# Autodesk Inventor assembly: Cover with Module - V1
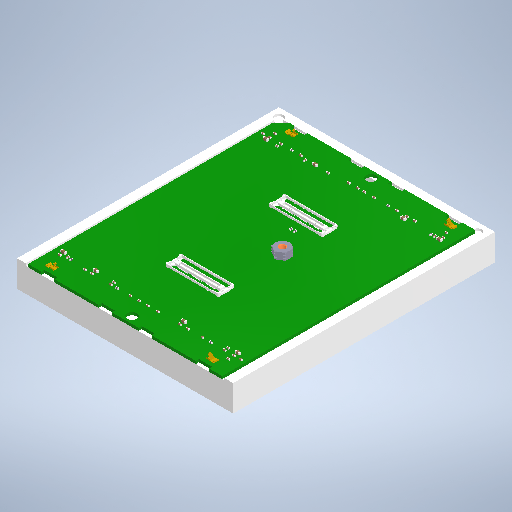
[picture p0: Inventor's stored thumbnail of the model, 512x512]
Saved by Autodesk Inventor 2025 (Build 290162000, 162)
## iProperties
Created: 2024-01-23
Part Number: Cover with Module - V1
Document SubType Name: Assembly
Designer: cfang
Author: cfang
## Documents named in this file (4)
- C:\Users\cfang\Desktop\nebraska-silicon-lab\Hardware\ETL\Module Assembly\Digital Module Cover - V1\Cover with Module - V1.iam
- C:\Users\cfang\Desktop\nebraska-silicon-lab\Hardware\ETL\modules\tamale v1.5\Tamale - V1p5p2.iam
- C:\Users\cfang\Desktop\nebraska-silicon-lab\Hardware\ETL\Module Assembly\Digital Module Cover - V1\Digital Module Cover - V1.ipt
- C:\Users\cfang\Desktop\nebraska-silicon-lab\Hardware\ETL\Module Assembly\Digital Module Cover - V1\Heat Sink - V1.ipt
## Components (3 placed, 3 different names)
1. Tamale - V1p5p2:1 [sub-assembly] — Mate:1, Angle:1, Mate:3, Mate:6
2. Digital Module Cover - V1:1 — Mate:1, Angle:1, Mate:3, Mate:4, Mate:5, Flush:1, Mate:6
3. Heat Sink - V1:1 — Mate:4, Mate:5, Flush:1
## Relationships (7: Mate 5, Angle 1, Flush 1)
- Mate:1: Tamale - V1p5p2:1 ↔ Digital Module Cover - V1:1
- Angle:1 (0 deg): Tamale - V1p5p2:1 ↔ Digital Module Cover - V1:1
- Mate:3 (0.5 mm): Tamale - V1p5p2:1 ↔ Digital Module Cover - V1:1
- Mate:4 (0.25 mm): Digital Module Cover - V1:1 ↔ Heat Sink - V1:1
- Mate:5 (0.25 mm): Digital Module Cover - V1:1 ↔ Heat Sink - V1:1
- Flush:1: Digital Module Cover - V1:1 ↔ Heat Sink - V1:1
- Mate:6: Tamale - V1p5p2:1 ↔ Digital Module Cover - V1:1
